# Autodesk Inventor assembly: Junk
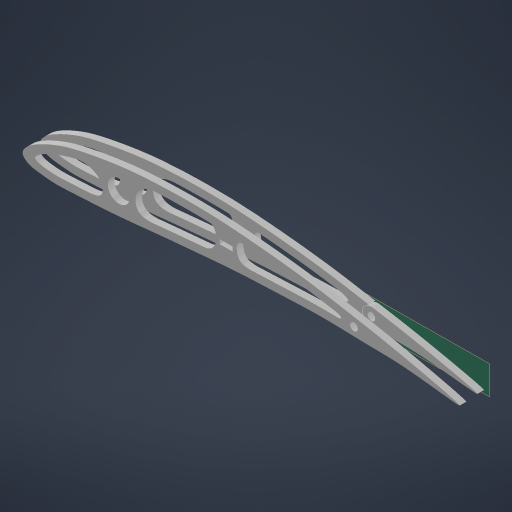
[picture p0: Inventor's stored thumbnail of the model, 512x512]
Saved by Autodesk Inventor 2023 (Build 270158000, 158)
## iProperties
Created: 2022-12-09
Part Number: Junk
Document SubType Name: Assembly
Designer: szykr
Author: szykr
## Documents named in this file (4)
- D:\Folder Instalacyjny\GitHub Pliki\Solaris\model\Junk.iam
- D:\Folder Instalacyjny\GitHub Pliki\Solaris\model\Żebro z lotką.ipt
- D:\Folder Instalacyjny\GitHub Pliki\Solaris\model\Lotka.ipt
- D:\Folder Instalacyjny\GitHub Pliki\Solaris\model\Żebro Default.ipt
## Components (3 placed, 3 different names)
1. Żebro z lotką:1 — Insert:1, Insert:2
2. Lotka:1 — Insert:1, Flush:1
3. Żebro Default:1 — Insert:2, Flush:1
## Relationships (3: Insert 2, Flush 1)
- Insert:1: Żebro z lotką:1 ↔ Lotka:1
- Insert:2 (5 mm): Żebro z lotką:1 ↔ Żebro Default:1
- Flush:1: Lotka:1 ↔ Żebro Default:1
